# Autodesk Inventor assembly: dnf3030_desk
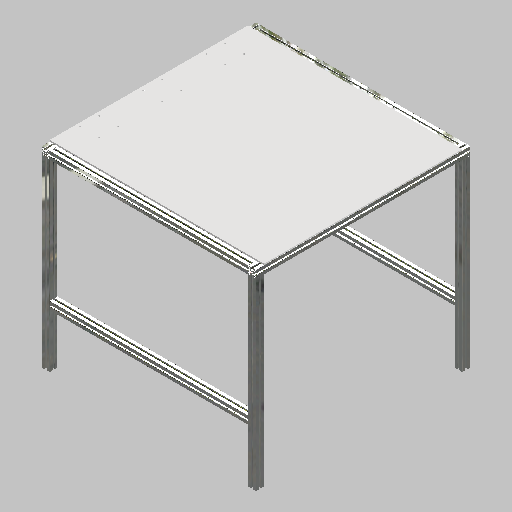
[picture p0: Inventor's stored thumbnail of the model, 512x512]
Saved by Autodesk Inventor 2026.2 (Build 302298000, 298)
## iProperties
Created: 2026-02-25
Part Number: dnf3030_desk
Document SubType Name: Assembly
Designer: mjbhang
Author: mjbhang
## Documents named in this file (5)
- C:\Users\mjbhang\Desktop\대학원\2025 소재부품기술개발사업-패키지형\robot_testbed\cad\dnf3030_base.iam
- C:\Users\mjbhang\Desktop\대학원\2025 소재부품기술개발사업-패키지형\robot_testbed\cad\profile\dnf3030\dnf3030_800.ipt
- C:\Users\mjbhang\Desktop\대학원\2025 소재부품기술개발사업-패키지형\robot_testbed\cad\profile\dnf3030\dnf3030_740.ipt
- C:\Users\mjbhang\Desktop\대학원\2025 소재부품기술개발사업-패키지형\robot_testbed\cad\profile\dnf3030\dnf3030_685.ipt
- C:\Users\mjbhang\Desktop\대학원\2025 소재부품기술개발사업-패키지형\robot_testbed\cad\plate\plate2.ipt
## Components (13 placed, 4 different names)
1. dnf3030_800:1 — 플러쉬:5, 메이트:3, 플러쉬:6, 플러쉬:7, 플러쉬:8, 메이트:4, 플러쉬:10, 메이트:6, 플러쉬:11, 플러쉬:12, 메이트:9, 플러쉬:17, 플러쉬:18
2. dnf3030_800:2 — 플러쉬:3, 플러쉬:4, 메이트:2, 메이트:7, 플러쉬:13, 플러쉬:14, 메이트:8, 플러쉬:15, 플러쉬:16, 메이트:11, 플러쉬:24, 메이트:14
3. dnf3030_740:1 — 플러쉬:3, 플러쉬:4, 메이트:2, 플러쉬:5, 메이트:3, 플러쉬:6, 플러쉬:25
4. dnf3030_740:2 — 플러쉬:7, 플러쉬:8, 메이트:4, 플러쉬:9, 메이트:5, 메이트:10, 플러쉬:19
5. dnf3030_740:3 — 플러쉬:9, 메이트:5, 플러쉬:10
6. dnf3030_685:1 — 메이트:7, 플러쉬:13, 플러쉬:14, 플러쉬:23
7. dnf3030_685:2 — 메이트:6, 플러쉬:11, 플러쉬:12, 메이트:13, 플러쉬:22
8. dnf3030_685:3 — 메이트:9, 플러쉬:17, 플러쉬:18, 메이트:12, 플러쉬:20, 플러쉬:21
9. dnf3030_685:4 — 메이트:8, 플러쉬:15, 플러쉬:16
10. dnf3030_740:4 — 메이트:10, 플러쉬:19, 메이트:11
11. dnf3030_740:5 — 메이트:12, 플러쉬:20, 플러쉬:21
12. dnf3030_740:6 — 메이트:13, 플러쉬:22, 플러쉬:23
13. plate2:1 — 플러쉬:24, 메이트:14, 플러쉬:25
## Relationships (36: Flush 23, Mate 13)
- 플러쉬:3 [Flush]: dnf3030_800:2 ↔ dnf3030_740:1
- 플러쉬:4 [Flush]: dnf3030_800:2 ↔ dnf3030_740:1
- 메이트:2 [Mate]: dnf3030_800:2 ↔ dnf3030_740:1
- 플러쉬:5 [Flush]: dnf3030_800:1 ↔ dnf3030_740:1
- 메이트:3 [Mate]: dnf3030_800:1 ↔ dnf3030_740:1
- 플러쉬:6 [Flush]: dnf3030_800:1 ↔ dnf3030_740:1
- 플러쉬:7 [Flush]: dnf3030_800:1 ↔ dnf3030_740:2
- 플러쉬:8 [Flush]: dnf3030_800:1 ↔ dnf3030_740:2
- 메이트:4 [Mate]: dnf3030_800:1 ↔ dnf3030_740:2
- 플러쉬:9 [Flush]: dnf3030_740:2 ↔ dnf3030_740:3
- 메이트:5 [Mate]: dnf3030_740:2 ↔ dnf3030_740:3
- 플러쉬:10 [Flush] (-230 mm): dnf3030_800:1 ↔ dnf3030_740:3
- 메이트:6 [Mate]: dnf3030_800:1 ↔ dnf3030_685:2
- 플러쉬:11 [Flush]: dnf3030_800:1 ↔ dnf3030_685:2
- 플러쉬:12 [Flush]: dnf3030_800:1 ↔ dnf3030_685:2
- 메이트:7 [Mate]: dnf3030_800:2 ↔ dnf3030_685:1
- 플러쉬:13 [Flush]: dnf3030_800:2 ↔ dnf3030_685:1
- 플러쉬:14 [Flush]: dnf3030_800:2 ↔ dnf3030_685:1
- 메이트:8 [Mate]: dnf3030_800:2 ↔ dnf3030_685:4
- 플러쉬:15 [Flush]: dnf3030_800:2 ↔ dnf3030_685:4
- 플러쉬:16 [Flush]: dnf3030_800:2 ↔ dnf3030_685:4
- 메이트:9 [Mate]: dnf3030_800:1 ↔ dnf3030_685:3
- 플러쉬:17 [Flush]: dnf3030_800:1 ↔ dnf3030_685:3
- 플러쉬:18 [Flush]: dnf3030_800:1 ↔ dnf3030_685:3
- 메이트:10 [Mate]: dnf3030_740:2 ↔ dnf3030_740:4
- 플러쉬:19 [Flush]: dnf3030_740:2 ↔ dnf3030_740:4
- 메이트:11 [Mate] (200 mm): dnf3030_800:2 ↔ dnf3030_740:4
- 메이트:12 [Mate]: dnf3030_685:3 ↔ dnf3030_740:5
- 플러쉬:20 [Flush]: dnf3030_685:3 ↔ dnf3030_740:5
- 플러쉬:21 [Flush] (-200 mm): dnf3030_685:3 ↔ dnf3030_740:5
- 메이트:13 [Mate]: dnf3030_685:2 ↔ dnf3030_740:6
- 플러쉬:22 [Flush]: dnf3030_685:2 ↔ dnf3030_740:6
- 플러쉬:23 [Flush] (-200 mm): dnf3030_685:1 ↔ dnf3030_740:6
- 플러쉬:24 [Flush]: dnf3030_800:2 ↔ plate2:1
- 메이트:14 [Mate]: dnf3030_800:2 ↔ plate2:1
- 플러쉬:25 [Flush] (30 mm): dnf3030_740:1 ↔ plate2:1
